# Autodesk Inventor assembly: roda
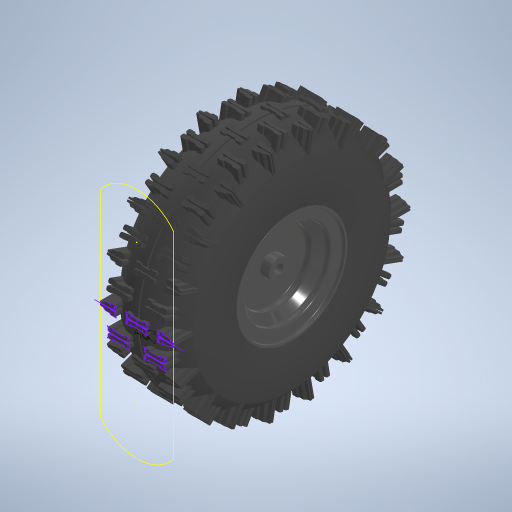
[picture p0: Inventor's stored thumbnail of the model, 512x512]
Saved by Autodesk Inventor 2023 (Build 270158000, 158)
## iProperties
Created: 2023-09-03
Part Number: roda
Document SubType Name: Assembly
Designer: sigit
Author: sigit
## Documents named in this file (4)
- D:\Kuliah\SEMESTER 7\Robot Semprot\Design\2nd ROBOT\Assembly\roda.iam
- D:\Kuliah\SEMESTER 7\Robot Semprot\Design\REVISI2\Part\ban.ipt
- D:\Kuliah\SEMESTER 7\Robot Semprot\Design\REVISI2\Part\velg.ipt
- D:\Kuliah\SEMESTER 7\Robot Semprot\Design\REVISI2\Part\sprocket\Roller Chain Sprocket64.ipt
## Components (3 placed, 3 different names)
1. ban:1 — Rotational:1
2. velg:1 — Rotational:1, Rotational:2
3. Roller Chain Sprocket2:1 — Rotational:2
## Relationships (2: RevoluteJoint 2)
- Rotational:1 [RevoluteJoint]: ban:1 ↔ velg:1
- Rotational:2 [RevoluteJoint]: velg:1 ↔ Roller Chain Sprocket2:1
